# Autodesk Inventor assembly: Assembly Base
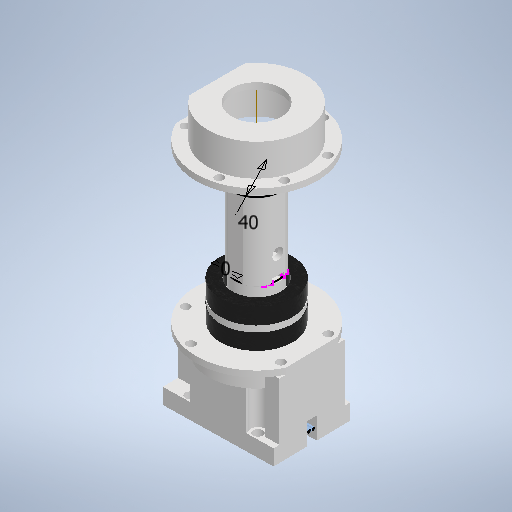
[picture p0: Inventor's stored thumbnail of the model, 512x512]
Saved by Autodesk Inventor 2025 (Build 290162000, 162)
## iProperties
Created: 2025-01-18
Part Number: Assembly Base
Document SubType Name: Assembly
Designer: Pauline Simonnet
Author: Pauline Simonnet
## Documents named in this file (6)
- C:\Users\Pauline Simonnet\Documents\ISAE SUPAERO\SupaeroMoon\MDRS\robotic arm\Assembly Base.iam
- C:\Users\Pauline Simonnet\Documents\ISAE SUPAERO\SupaeroMoon\MDRS\robotic arm\B2.ipt
- C:\Users\Pauline Simonnet\Documents\ISAE SUPAERO\SupaeroMoon\MDRS\robotic arm\Base\B1.ipt
- C:\Users\Pauline Simonnet\Documents\ISAE SUPAERO\SupaeroMoon\MDRS\robotic arm\Base\B1 fixe2.ipt
- C:\Users\Pauline Simonnet\Documents\ISAE SUPAERO\SupaeroMoon\MDRS\components\bearings base.ipt
- C:\Users\Pauline Simonnet\Documents\ISAE SUPAERO\SupaeroMoon\MDRS\components\motor_25kg.iam
## Components (6 placed, 5 different names)
1. B2:1 — Mate:1, Mate:3, Mate:4, Mate:8, Mate:9
2. B1:1 — Mate:1, Mate:2, Mate:5, Mate:6, Mate:10
3. B1 fixe2:1 — Mate:2
4. bearings base:1 — Mate:3, Mate:8, Mate:10
5. bearings base:2 — Mate:4, Mate:9
6. motor_25kg:1 [sub-assembly] — Mate:5, Mate:6
## Relationships (9: Mate 9)
- Mate:1: B2:1 ↔ B1:1
- Mate:2: B1:1 ↔ B1 fixe2:1
- Mate:3: B2:1 ↔ bearings base:1
- Mate:4: B2:1 ↔ bearings base:2
- Mate:5: B1:1 ↔ motor_25kg:1
- Mate:6: B1:1 ↔ motor_25kg:1
- Mate:8: B2:1 ↔ bearings base:1
- Mate:9: B2:1 ↔ bearings base:2
- Mate:10: B1:1 ↔ bearings base:1
